# Autodesk Inventor assembly: gear-stack-enormous
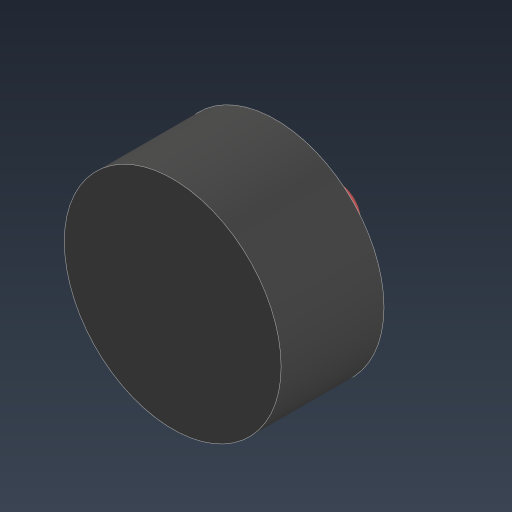
[picture p0: Inventor's stored thumbnail of the model, 512x512]
Saved by Autodesk Inventor 2023 (Build 270158000, 158)
## iProperties
Created: 2025-04-27
Part Number: gear-stack-enormous
Document SubType Name: Assembly
Designer: szymo
Mass: 12 g
Surface Area: 96.3848 cm^2
Volume: 23.0778 cm^3
Density: 0.519981 g/cm^3
Author: szymo
## Documents named in this file (8)
- D:\tech\robotyka\robots\evangelion\inventor-project\gear-stack-enormous.iam
- D:\tech\robotyka\robots\evangelion\inventor-project\gear-stack-enormous\Design Accelerator\Spur Gears1.iam
- D:\tech\robotyka\robots\evangelion\inventor-project\Shaft1.ipt
- D:\tech\robotyka\robots\evangelion\inventor-project\wheel.ipt
- D:\tech\robotyka\robots\evangelion\inventor-project\oponka.ipt
- D:\tech\robotyka\robots\evangelion\inventor-project\ball-bearing.ipt
- D:\tech\robotyka\robots\evangelion\inventor-project\bearing SF-1F-8mm.ipt
- D:\tech\robotyka\robots\evangelion\inventor-project\hold-fur-wylewanko.ipt
## Components (7 placed, 7 different names)
1. Spur Gears:1 [sub-assembly] — Mate:1, Mate:2, Mate:3, Mate:8, Mate:9, Flush:1, Angle:1, Angle:2, Angle:3, Mate:14, Mate:16
2. Shaft:1 — Mate:1, Mate:2, Mate:3, Mate:10, Mate:12, Mate:15
3. wheel:1 — Mate:10, Flush:2, Flush:3
4. oponka:1 — Flush:2
5. ball-bearing:2 — Mate:12, Mate:14
6. bearing SF-1F-8mm:1 — Mate:15, Mate:16
7. hold-fur-wylewanko:1 — Flush:3
## Relationships (16: Mate 10, Flush 3, Angle 3)
- Mate:1: Spur Gears:1 ↔ Shaft:1
- Mate:2: Spur Gears:1 ↔ Shaft:1
- Mate:3: Spur Gears:1 ↔ Shaft:1
- Mate:8: Spur Gears:1
- Mate:9: Spur Gears:1
- Flush:1: Spur Gears:1
- Angle:1 (180 deg): Spur Gears:1
- Angle:2 (180 deg): Spur Gears:1
- Angle:3 (0 deg): Spur Gears:1
- Mate:10: Shaft:1 ↔ wheel:1
- Flush:2: wheel:1 ↔ oponka:1
- Mate:12: Shaft:1 ↔ ball-bearing:2
- Mate:14 (0.4 mm): Spur Gears:1 ↔ ball-bearing:2
- Mate:15: Shaft:1 ↔ bearing SF-1F-8mm:1
- Mate:16 (0.1 mm): Spur Gears:1 ↔ bearing SF-1F-8mm:1
- Flush:3: wheel:1 ↔ hold-fur-wylewanko:1
